# Autodesk Inventor assembly: Drive
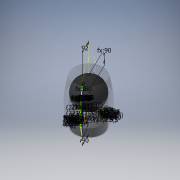
[picture p0: Inventor's stored thumbnail of the model, 180x180]
Saved by Autodesk Inventor 2018.3 (Build 223284000, 284)
## iProperties
Created: 2018-06-30
Part Number: Drive
Material: Generisch
Document SubType Name: Assembly
Designer: JochenAlt
Author: JochenAlt
## Documents named in this file (4)
- D:\Projects\FlowerPot\CAD\Drive.iam
- D:\Projects\FlowerPot\CAD\DriveChain.iam
- D:\Projects\FlowerPot\CAD\Sphere.ipt
- D:\Projects\FlowerPot\CAD\Form.ipt
## Components (5 placed, 3 different names)
1. Antriebsstrang:1 [sub-assembly] — Passend:1, Passend:3, Passend:5, Tangential:1, Passend:6, Passend:8, Passend:9
2. Antriebsstrang:2 [sub-assembly] — Passend:2, Passend:4, Passend:6, Passend:7, Passend:11
3. Antriebsstrang:3 [sub-assembly] — Passend:1, Passend:2, Passend:3, Passend:4, Passend:7, Passend:8
4. Sphere:1 — Passend:5, Tangential:1
5. Form:1 — Passend:9, Passend:10, Passend:11
## Relationships (12: Mate 11, Tangent 1)
- Passend:1 [Mate]: Antriebsstrang:1 ↔ Antriebsstrang:3
- Passend:2 [Mate]: Antriebsstrang:2 ↔ Antriebsstrang:3
- Passend:3 [Mate]: Antriebsstrang:1 ↔ Antriebsstrang:3
- Passend:4 [Mate]: Antriebsstrang:2 ↔ Antriebsstrang:3
- Passend:5 [Mate]: Antriebsstrang:1 ↔ Sphere:1
- Tangential:1: Antriebsstrang:1 ↔ Sphere:1
- Passend:6 [Mate]: Antriebsstrang:1 ↔ Antriebsstrang:2
- Passend:7 [Mate]: Antriebsstrang:2 ↔ Antriebsstrang:3
- Passend:8 [Mate]: Antriebsstrang:1 ↔ Antriebsstrang:3
- Passend:9 [Mate]: Antriebsstrang:1 ↔ Form:1
- Passend:10 [Mate]: Form:1
- Passend:11 [Mate]: Antriebsstrang:2 ↔ Form:1
